# Autodesk Inventor assembly: a ball end
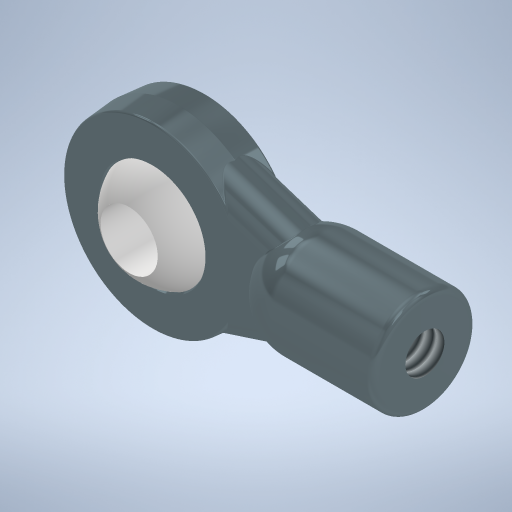
[picture p0: Inventor's stored thumbnail of the model, 512x512]
Saved by Autodesk Inventor 2024 (Build 280153000, 153)
## iProperties
Created: 2023-07-07
Part Number: a ball end
Document SubType Name: Assembly
Designer: birud
Author: birud
## Documents named in this file (3)
- C:\Users\birud\OneDrive\Desktop\Openers\a ball end.iam
- C:\Users\birud\OneDrive\Desktop\Openers\SA Ball End.ipt
- C:\Users\birud\OneDrive\Desktop\Openers\ball.ipt
## Components (2 placed, 2 different names)
1. SA Ball End:1 — Mate:1, Mate:2
2. ball:1 — Mate:1, Mate:2
## Relationships (2: Mate 2)
- Mate:1: SA Ball End:1 ↔ ball:1
- Mate:2: SA Ball End:1 ↔ ball:1
